# Autodesk Inventor assembly: Radiation Sheild
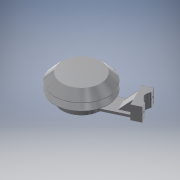
[picture p0: Inventor's stored thumbnail of the model, 180x180]
Saved by Autodesk Inventor 2019 (Build 230136000, 136)
## iProperties
Created: 2020-02-28
Part Number: Radiation Sheild
Document SubType Name: Assembly
Designer: gfb14170
Author: gfb14170
## Documents named in this file (5)
- N:\Sandpit\Callum Brooksby\Radiation Sheild\Radiation Sheild.iam
- N:\Sandpit\Callum Brooksby\Radiation Sheild\Rad_Shd_Base_V1.ipt
- N:\Sandpit\Callum Brooksby\Radiation Sheild\Rad_Shd_Vert_mount_V1.ipt
- N:\Sandpit\Callum Brooksby\Radiation Sheild\Rad_Shd_Fin_V1.ipt
- N:\Sandpit\Callum Brooksby\Radiation Sheild\Rad_Shd_Top_V1.ipt
## Components (4 placed, 4 different names)
1. Rad_Shd_Base_V1:1 — Insert:4
2. Rad_Shd_Vert_mount_V1:1
3. Rad_Shd_Fin_V1:1 — Insert:3, Insert:4
4. Rad_Shd_Top_V1:1 — Insert:3
## Relationships (2: Insert 2)
- Insert:3 (-401 mm): Rad_Shd_Fin_V1:1 ↔ Rad_Shd_Top_V1:1
- Insert:4 (-290 mm): Rad_Shd_Base_V1:1 ↔ Rad_Shd_Fin_V1:1
